# Autodesk Inventor assembly: 739136
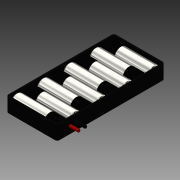
[picture p0: Inventor's stored thumbnail of the model, 180x180]
Saved by Autodesk Inventor 2016 SP1 (Build 200210100, 210)
## iProperties
Category: Electrical Accessories
Company: Autodesk Inc.
Created: 2014-11-27
Part Number: 739136
Document SubType Name: Assembly
Designer: Tetrix
Catalog Web Link: http://www.tetrixrobotics.com/AA_Battery_Holder
Vendor: Tetrix
Author: Autodesk Inc.
## Documents named in this file (3)
- D:\FIRST\FTC\FTC KOP 2016\Tetrix\Tetrix_739136.iam
- D:\FIRST\FTC\FTC KOP 2016\Tetrix\Tetrix_739136_Holder.ipt
- D:\FIRST\FTC\FTC KOP 2016\Tetrix\Tetrix_739136_AA.ipt
## Components (9 placed, 2 different names)
1. Tetrix_739136_Holder:1 — Tangent:1, Mate:1, Tangent:2, Tangent:3, Tangent:4, Mate:2
2. Tetrix_739136_AA:2 — Tangent:3, Tangent:4, Mate:2
3. Tetrix_739136_AA:3
4. Tetrix_739136_AA:4
5. Tetrix_739136_AA:5
6. Tetrix_739136_AA:1 — Tangent:1, Mate:1, Tangent:2
7. Tetrix_739136_AA:6
8. Tetrix_739136_AA:7
9. Tetrix_739136_AA:8
## Component patterns: (4 elements, first: Tetrix_739136_AA:2), (4 elements, first: Tetrix_739136_AA:1)
## Relationships (6: Tangent 4, Mate 2)
- Tangent:1: Tetrix_739136_Holder:1 ↔ Tetrix_739136_AA:1
- Mate:1: Tetrix_739136_Holder:1 ↔ Tetrix_739136_AA:1
- Tangent:2: Tetrix_739136_Holder:1 ↔ Tetrix_739136_AA:1
- Tangent:3: Tetrix_739136_Holder:1 ↔ Tetrix_739136_AA:2
- Tangent:4: Tetrix_739136_Holder:1 ↔ Tetrix_739136_AA:2
- Mate:2: Tetrix_739136_Holder:1 ↔ Tetrix_739136_AA:2
